# Autodesk Inventor assembly: VersaPlanetary_Lite_0_Stage_3_8_Hex
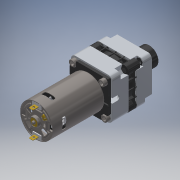
[picture p0: Inventor's stored thumbnail of the model, 180x180]
Saved by Autodesk Inventor 2018 (Build 220112000, 112)
## iProperties
Created: 2017-12-05
Part Number: VersaPlanetary_Lite_0_Stage_3_8_Hex
Description: STEP AP214
Document SubType Name: Assembly
Designer: maste
Sending System: SolidWorks 2017
Preprocessor: SwSTEP 2.0
Title: VersaPlanetary-Lite-0-Stage-NeveRest-20171205.STEP
Revision Number: ANY
## Documents named in this file (10)
- C:\Users\maste\OneDrive\Documents\GitHub\2020CAD\Control panel spinny boi\Part Files\VersaPlanetary_Lite_0_Stage_3_8_Hex.iam
- C:\Users\maste\OneDrive\Documents\GitHub\2020CAD\Control panel spinny boi\Part Files\VersaPlanetary Output Blocks_VP Lite Output Block.iam
- C:\Users\maste\OneDrive\Documents\GitHub\2020CAD\Control panel spinny boi\Part Files\VersaPlanetary Output Shafts_0.375_ Hex (217-2625-021).iam
- C:\Users\maste\OneDrive\Documents\GitHub\2020CAD\Control panel spinny boi\Part Files\217-2625-018 Rev1_98541A410.ipt
- C:\Users\maste\OneDrive\Documents\GitHub\2020CAD\Control panel spinny boi\Part Files\VersaPlanetary Input Blocks_VP LIte Input Block.iam
- C:\Users\maste\OneDrive\Documents\GitHub\2020CAD\Control panel spinny boi\Part Files\VersaPlanetary All Non-CIM Motors_NeveRest Motor.iam
- C:\Users\maste\OneDrive\Documents\GitHub\2020CAD\Control panel spinny boi\Part Files\#8-32 SHCS, Grade 8 Steel Rev2_SSA0832-0500ZB.ipt
- C:\Users\maste\OneDrive\Documents\GitHub\2020CAD\Control panel spinny boi\Part Files\#8-32 SHCS, Grade 8 Steel Rev2_SSA0832-1125ZB.ipt
- C:\Users\maste\OneDrive\Documents\GitHub\2020CAD\Control panel spinny boi\Part Files\VersaPlanetary_Lite_Ring_Gear.ipt
- C:\Users\maste\OneDrive\Documents\GitHub\2020CAD\Control panel spinny boi\Part Files\Universal_Female_Output_Shaft_1_2_Hex.ipt
## Components (11 placed, 11 different names)
1. VersaPlanetary Output Blocks_VP Lite Output Block_1 [sub-assembly] — Mate:4, Rotation:2, Mate:7, Mate:9
2. VersaPlanetary Output Shafts_0.375" Hex (217-2625-021)_2 [sub-assembly] — Mate:4
3. 217-2625-018 Rev1_98541A410_3 — Mate:8
4. VersaPlanetary Input Blocks_VP LIte Input Block_4 [sub-assembly] — Rotation:2, Mate:5, Mate:6
5. VersaPlanetary All Non-CIM Motors_NeveRest Motor_5 [sub-assembly]
6. #8-32 SHCS, Grade 8 Steel Rev2_SSA0832-0500ZB_6
7. #8-32 SHCS, Grade 8 Steel Rev2_SSA0832-0500ZB_7
8. #8-32 SHCS, Grade 8 Steel Rev2_SSA0832-1125ZB_8
9. #8-32 SHCS, Grade 8 Steel Rev2_SSA0832-1125ZB_9
10. VersaPlanetary_Lite_Ring_Gear:1 — Mate:5, Mate:6, Mate:7
11. Universal_Female_Output_Shaft_1_2_Hex:1 — Mate:8, Mate:9
## Relationships (7: Mate 6, RelateRotation 1)
- Mate:4: VersaPlanetary Output Blocks_VP Lite Output Block_1 ↔ VersaPlanetary Output Shafts_0.375" Hex (217-2625-021)_2
- Rotation:2 [RelateRotation] (1 ul): VersaPlanetary Output Blocks_VP Lite Output Block_1 ↔ VersaPlanetary Input Blocks_VP LIte Input Block_4
- Mate:5: VersaPlanetary Input Blocks_VP LIte Input Block_4 ↔ VersaPlanetary_Lite_Ring_Gear:1
- Mate:6: VersaPlanetary Input Blocks_VP LIte Input Block_4 ↔ VersaPlanetary_Lite_Ring_Gear:1
- Mate:7: VersaPlanetary Output Blocks_VP Lite Output Block_1 ↔ VersaPlanetary_Lite_Ring_Gear:1
- Mate:8: 217-2625-018 Rev1_98541A410_3 ↔ Universal_Female_Output_Shaft_1_2_Hex:1
- Mate:9: VersaPlanetary Output Blocks_VP Lite Output Block_1 ↔ Universal_Female_Output_Shaft_1_2_Hex:1
